# Autodesk Inventor assembly: Surub M3 25
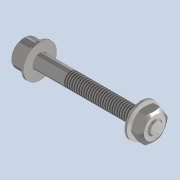
[picture p0: Inventor's stored thumbnail of the model, 180x180]
Saved by Autodesk Inventor 2020 (Build 240168000, 168)
## iProperties
Created: 2020-12-21
Part Number: Surub M3 25
Document SubType Name: Assembly
Designer: Iulian Bors
Author: Iulian Bors
## Documents named in this file (4)
- Z:\I.A.B\Proiecte\0005 I.A.B 3d 2.0 Imprimanta aracet\10 Mecanic\Surub M3 25.iam
- Z:\I.A.B\Proiecte\0005 I.A.B 3d 2.0 Imprimanta aracet\10 Mecanic\0005-10-1020 ISO 7089 - 3 - 140 HV(1).ipt
- Z:\I.A.B\Proiecte\0005 I.A.B 3d 2.0 Imprimanta aracet\10 Mecanic\0005-10-1021 ISO 4032 - M3 - ISO.ipt
- Z:\I.A.B\Proiecte\0005 I.A.B 3d 2.0 Imprimanta aracet\10 Mecanic\0005-10-1053 ISO 4762 - M3 x 25.ipt
## Components (4 placed, 3 different names)
1. ISO 4762 - M3 x 25ISO.ipt:1 — Mate:1, Mate:2, Insert:1
2. 0005-10-1020 ISO 7089 - 3 - 140 HV(1).ipt:2 — Mate:1, Mate:2
3. 0005-10-1021 ISO 4032 - M3 - ISO.ipt:3 — Insert:1, Insert:2
4. 0005-10-1020 ISO 7089 - 3 - 140 HV(1).ipt:4 — Insert:2
## Relationships (4: Mate 2, Insert 2)
- Mate:1: ISO 4762 - M3 x 25ISO.ipt:1 ↔ 0005-10-1020 ISO 7089 - 3 - 140 HV(1).ipt:2
- Mate:2: ISO 4762 - M3 x 25ISO.ipt:1 ↔ 0005-10-1020 ISO 7089 - 3 - 140 HV(1).ipt:2
- Insert:1: ISO 4762 - M3 x 25ISO.ipt:1 ↔ 0005-10-1021 ISO 4032 - M3 - ISO.ipt:3
- Insert:2: 0005-10-1021 ISO 4032 - M3 - ISO.ipt:3 ↔ 0005-10-1020 ISO 7089 - 3 - 140 HV(1).ipt:4
